# Autodesk Inventor assembly: ServoMotor_CaseTH_Interno
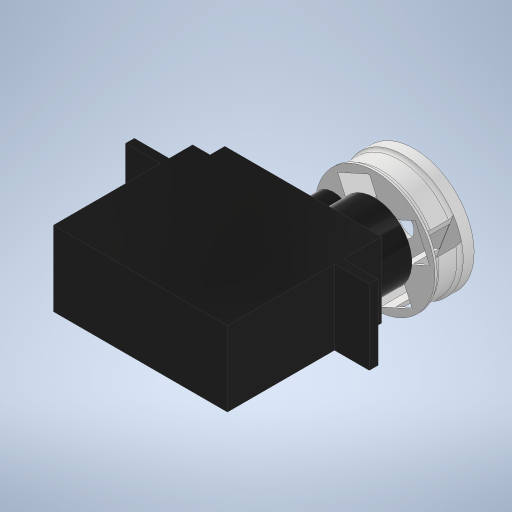
[picture p0: Inventor's stored thumbnail of the model, 512x512]
Saved by Autodesk Inventor 2024.2 (Build 282272000, 272)
## iProperties
Created: 2023-10-04
Part Number: ServoMotor_CaseTH_Interno
Document SubType Name: Assembly
Designer: Alexander Saavedra
Author: Alexander Saavedra
## Documents named in this file (4)
- C:\Users\Laboratorio IA\Documents\handi-epn\CAD\purchased components (motors, magnets, screws, electronics)\servoMotor\ServoMotor_CaseTH_Interno.iam
- C:\Users\Laboratorio IA\Documents\handi-epn\CAD\purchased components (motors, magnets, screws, electronics)\servoMotor\Servo.ipt
- C:\Users\Laboratorio IA\Documents\handi-epn\CAD\purchased components (motors, magnets, screws, electronics)\servoMotor\Servo Spool Thumb.ipt
- C:\Users\Laboratorio IA\Documents\handi-epn\CAD\purchased components (motors, magnets, screws, electronics)\Servo Spool D2-3-4_HS40.ipt
## Components (3 placed, 3 different names)
1. Servo:1 — Insert:1, Rotational:1
2. Servo Spool Thumb:1 — Rotational:1
3. Servo Spool D2-3-4_HS40:1 — Insert:1
## Relationships (2: Insert 1, RevoluteJoint 1)
- Insert:1 (3.7 mm): Servo:1 ↔ Servo Spool D2-3-4_HS40:1
- Rotational:1 [RevoluteJoint] (3.25 mm): Servo:1 ↔ Servo Spool Thumb:1
